# Autodesk Inventor assembly: x-IMU 2 Housing
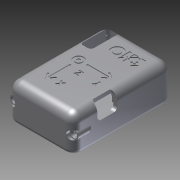
[picture p0: Inventor's stored thumbnail of the model, 180x180]
Saved by Autodesk Inventor 2011 (Build 150239000, 239)
## iProperties
Created: 2011-08-18
Part Number: x-IMU 2 Housing
Document SubType Name: Assembly
Designer: Jacky
Author: Jacky
## Documents named in this file (3)
- C:\MyFiles\x-io\Products\x-IMU\x-IMU-Housing\x-IMU Housing.iam
- C:\MyFiles\x-io\Products\x-IMU\x-IMU-Housing\x-IMU Housing Main.ipt
- C:\MyFiles\x-io\Products\x-IMU\x-IMU-Housing\x-IMU Housing Lid.ipt
## Components (2 placed, 2 different names)
1. x-IMU Housing Main:1 — Insert:1, Insert:2
2. x-IMU Housing Lid:1 — Insert:1, Insert:2
## Relationships (2: Insert 2)
- Insert:1: x-IMU Housing Main:1 ↔ x-IMU Housing Lid:1
- Insert:2: x-IMU Housing Main:1 ↔ x-IMU Housing Lid:1
